# Autodesk Inventor assembly: Kit Frame 24x32
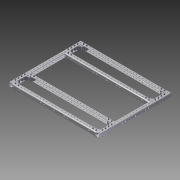
[picture p0: Inventor's stored thumbnail of the model, 180x180]
Saved by Autodesk Inventor 2013 (Build 170138000, 138)
## iProperties
Created: 2013-01-06
Part Number: Kit Frame 24x32
Document SubType Name: Assembly
Designer: Nemo
Author: Nemo
## Documents named in this file (4)
- \\lmss\students\Robotics\CAD Files\COTS Parts\Kit Frame - AndyMark\Kit Frame 24x32.iam
- \\lmss\students\Robotics\CAD Files\COTS Parts\Kit Frame - AndyMark\Components\24x34 Side Rail sub.iam
- \\lmss\students\Robotics\CAD Files\COTS Parts\Kit Frame - AndyMark\Components\24x32 Side Rail Sub mirror.iam
- \\lmss\students\Robotics\CAD Files\COTS Parts\Kit Frame - AndyMark\Components\C Channel - FrontBack 24x32.ipt
## Components (6 placed, 3 different names)
1. C Channel - Cut-01:3 — Flush:5
2. C Channel - Cut-01:4 — Mate:3, Insert:5, Mate:11, Insert:6, Mate:12
3. 24x34 Side Rail sub:1 [sub-assembly]
4. 24x34 Side Rail sub:2 [sub-assembly] — Insert:5, Mate:11
5. 24x32 Side Rail Sub mirror:1 [sub-assembly]
6. 24x32 Side Rail Sub mirror:2 [sub-assembly] — Insert:6, Mate:12
## Relationships (19: Mate 8, Insert 6, Flush 5)
- [Mate] (36.83 mm): 24x34 Side Rail sub:1
- [Flush]: 24x34 Side Rail sub:1 ↔ 24x32 Side Rail Sub mirror:1
- [Mate]: 24x34 Side Rail sub:1
- [Flush]: 24x32 Side Rail Sub mirror:1
- [Flush]: C Channel - Cut-01:3 ↔ 24x34 Side Rail sub:1
- [Flush]: C Channel - Cut-01:4 ↔ 24x34 Side Rail sub:1
- Flush:5: C Channel - Cut-01:3
- Mate:3: C Channel - Cut-01:4
- [Insert]: C Channel - Cut-01:4 ↔ 24x34 Side Rail sub:1
- [Insert]: C Channel - Cut-01:4 ↔ 24x32 Side Rail Sub mirror:1
- [Mate]: C Channel - Cut-01:4 ↔ 24x32 Side Rail Sub mirror:1
- [Insert]: C Channel - Cut-01:3 ↔ 24x34 Side Rail sub:1
- [Mate]: C Channel - Cut-01:3 ↔ 24x34 Side Rail sub:1
- [Insert]: C Channel - Cut-01:3 ↔ 24x32 Side Rail Sub mirror:1
- [Mate]: C Channel - Cut-01:3 ↔ 24x32 Side Rail Sub mirror:1
- Insert:5: C Channel - Cut-01:4 ↔ 24x34 Side Rail sub:2
- Mate:11: C Channel - Cut-01:4 ↔ 24x34 Side Rail sub:2
- Insert:6: C Channel - Cut-01:4 ↔ 24x32 Side Rail Sub mirror:2
- Mate:12: C Channel - Cut-01:4 ↔ 24x32 Side Rail Sub mirror:2
